# Autodesk Inventor assembly: m4 bearing assembly
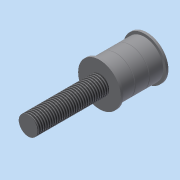
[picture p0: Inventor's stored thumbnail of the model, 180x180]
Saved by Autodesk Inventor 2015 (Build 190159000, 159)
## iProperties
Created: 2016-09-08
Part Number: m4 bearing assembly
Document SubType Name: Assembly
Designer: Dustin
Author: Dustin
## Documents named in this file (4)
- E:\Documents\3D Printer\LetzteBot3DPrinter\Inventor Files\IAM Files\m4 bearing assembly.iam
- E:\Documents\3D Printer\Parts\New Printer\m4x40.ipt
- E:\Documents\3D Printer\Parts\New Printer\8x4x3 bearing.ipt
- E:\Documents\3D Printer\Parts\New Printer\washer.ipt
## Components (6 placed, 3 different names)
1. m4x40:1 — Angle:1, Tangent:1, Mate:1, Angle:2, Tangent:2, Angle:3, Tangent:3, Insert:1
2. 8x4x3 bearing:1 — Angle:3, Tangent:3, Mate:3, Insert:2
3. 8x4x3 bearing:2 — Angle:2, Tangent:2, Mate:2, Mate:3
4. 8x4x3 bearing:3 — Angle:1, Tangent:1, Mate:1, Mate:2
5. washer:1 — Insert:1
6. washer:2 — Insert:2
## Relationships (11: Angle 3, Tangent 3, Mate 3, Insert 2)
- Angle:1 (0 deg): m4x40:1 ↔ 8x4x3 bearing:3
- Tangent:1: m4x40:1 ↔ 8x4x3 bearing:3
- Mate:1 (0.5 mm): m4x40:1 ↔ 8x4x3 bearing:3
- Angle:2 (0 deg): m4x40:1 ↔ 8x4x3 bearing:2
- Tangent:2: m4x40:1 ↔ 8x4x3 bearing:2
- Mate:2: 8x4x3 bearing:2 ↔ 8x4x3 bearing:3
- Angle:3 (0 deg): m4x40:1 ↔ 8x4x3 bearing:1
- Tangent:3: m4x40:1 ↔ 8x4x3 bearing:1
- Mate:3: 8x4x3 bearing:1 ↔ 8x4x3 bearing:2
- Insert:1: m4x40:1 ↔ washer:1
- Insert:2: 8x4x3 bearing:1 ↔ washer:2
